# Autodesk Inventor assembly: ChainlinkVP
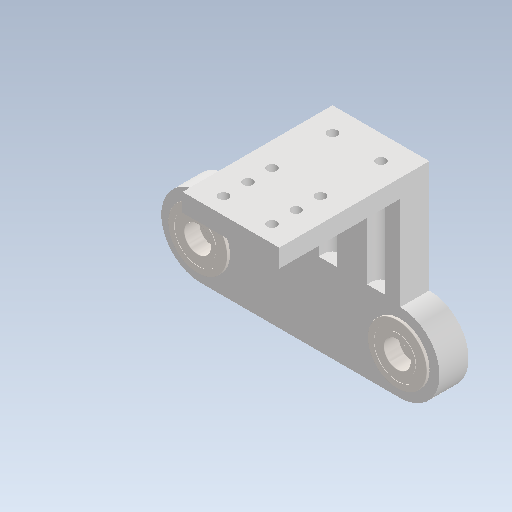
[picture p0: Inventor's stored thumbnail of the model, 512x512]
Saved by Autodesk Inventor 2020 (Build 240168000, 168)
## iProperties
Created: 2020-01-19
Part Number: ChainlinkVP
Document SubType Name: Assembly
Designer: srini
Author: srini
## Documents named in this file (3)
- C:\Users\srini\Documents\FRC\2020\IntakeShooter\ChainlinkVP.iam
- C:\Users\srini\Documents\FRC\2020\IntakeShooter\IntakeChainLinkVP.ipt
- C:\Users\srini\Documents\FRC\2020\IntakeShooter\13_75mm_1_2_ThunderHex_ID_x_1_125_OD_x_0_313_WD_Flanged_Bearing_217-4006.ipt
## Components (5 placed, 2 different names)
1. IntakeChainLinkVP:1 — Insert:1, Insert:2, Insert:3, Insert:4
2. 13_75mm_1_2_ThunderHex_ID_x_1_125_OD_x_0_313_WD_Flanged_Bearing_217-4006:1 — Insert:1
3. 13_75mm_1_2_ThunderHex_ID_x_1_125_OD_x_0_313_WD_Flanged_Bearing_217-4006:2 — Insert:4
4. 13_75mm_1_2_ThunderHex_ID_x_1_125_OD_x_0_313_WD_Flanged_Bearing_217-4006:3 — Insert:2
5. 13_75mm_1_2_ThunderHex_ID_x_1_125_OD_x_0_313_WD_Flanged_Bearing_217-4006:4 — Insert:3
## Relationships (4: Insert 4)
- Insert:1: IntakeChainLinkVP:1 ↔ 13_75mm_1_2_ThunderHex_ID_x_1_125_OD_x_0_313_WD_Flanged_Bearing_217-4006:1
- Insert:2: IntakeChainLinkVP:1 ↔ 13_75mm_1_2_ThunderHex_ID_x_1_125_OD_x_0_313_WD_Flanged_Bearing_217-4006:3
- Insert:3: IntakeChainLinkVP:1 ↔ 13_75mm_1_2_ThunderHex_ID_x_1_125_OD_x_0_313_WD_Flanged_Bearing_217-4006:4
- Insert:4: IntakeChainLinkVP:1 ↔ 13_75mm_1_2_ThunderHex_ID_x_1_125_OD_x_0_313_WD_Flanged_Bearing_217-4006:2
